# Autodesk Inventor assembly: brace
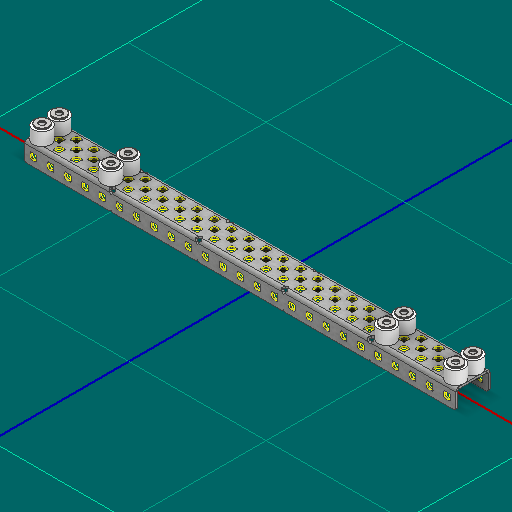
[picture p0: Inventor's stored thumbnail of the model, 512x512]
Saved by Autodesk Inventor 2025 (Build 290162000, 162)
## iProperties
Created: 2024-10-07
Part Number: brace
Document SubType Name: Assembly
Designer: averey
Author: averey
## Documents named in this file (7)
- C:\Users\avere\vex_robotics_high_stakes\hardware\cad\bots\high_stakes_v2\chassis\brace.iam
- C:\Users\avere\vex_robotics_high_stakes\hardware\cad\robpros_cad_lib\Structure\C Channel\Aluminum 1x2x1\Alu C 1x2x1x25.ipt
- C:\Users\avere\vex_robotics_high_stakes\hardware\cad\VEX-CAD-Inventor\Motion\Spacers\Spacer Nylon .500 OD\NSpacer White .500 OD x .375.ipt
- C:\Users\avere\vex_robotics_high_stakes\hardware\cad\VEX-CAD-Inventor\Motion\Spacers\Spacer Nylon .500 OD.ipt
- C:\Users\avere\vex_robotics_high_stakes\hardware\cad\VEX-CAD-Inventor\Motion\Spacers\Washer Steel\SWasher .375 OD x .031250.ipt
- C:\Users\avere\vex_robotics_high_stakes\hardware\cad\VEX-CAD-Inventor\Motion\Spacers\Washer Steel.ipt
- C:\Users\avere\vex_robotics_high_stakes\hardware\cad\VEX-CAD-Inventor\Motion\Spacers\Washer Steel\SWasher .375 OD x .015625.ipt
## Components (25 placed, 4 different names)
1. Alu C 1x2x1x25:1 — Mate:1, Insert:6, Insert:9, Insert:12, Insert:15, Insert:18, Insert:23, Insert:24
2. NSpacer White .500 OD x .375:1 — Insert:6
3. SWasher .375 OD x .031250:1
4. SWasher .375 OD x .015625:2
5. NSpacer White .500 OD x .375:2
6. SWasher .375 OD x .031250:3
7. SWasher .375 OD x .015625:4
8. NSpacer White .500 OD x .375:3 — Insert:9
9. SWasher .375 OD x .031250:5
10. SWasher .375 OD x .015625:6
11. NSpacer White .500 OD x .375:4 — Insert:12
12. SWasher .375 OD x .031250:7
13. SWasher .375 OD x .015625:8
14. NSpacer White .500 OD x .375:5 — Insert:15
15. SWasher .375 OD x .031250:9
16. SWasher .375 OD x .015625:10
17. NSpacer White .500 OD x .375:6 — Insert:18
18. SWasher .375 OD x .031250:11
19. SWasher .375 OD x .015625:12
20. NSpacer White .500 OD x .375:7 — Insert:24
21. SWasher .375 OD x .031250:13
22. SWasher .375 OD x .015625:14
23. NSpacer White .500 OD x .375:8 — Insert:23
24. SWasher .375 OD x .031250:15
25. SWasher .375 OD x .015625:16
## Relationships (25: Insert 24, Mate 1)
- [Insert]: NSpacer White .500 OD x .375:1 ↔ SWasher .375 OD x .031250:1
- [Insert]: SWasher .375 OD x .031250:1 ↔ SWasher .375 OD x .015625:2
- [Insert]: NSpacer White .500 OD x .375:2 ↔ SWasher .375 OD x .031250:3
- [Insert]: SWasher .375 OD x .031250:3 ↔ SWasher .375 OD x .015625:4
- [Insert]: Alu C 1x2x1x25:1 ↔ NSpacer White .500 OD x .375:2
- Mate:1: Alu C 1x2x1x25:1
- Insert:6: Alu C 1x2x1x25:1 ↔ NSpacer White .500 OD x .375:1
- [Insert]: NSpacer White .500 OD x .375:3 ↔ SWasher .375 OD x .031250:5
- [Insert]: SWasher .375 OD x .031250:5 ↔ SWasher .375 OD x .015625:6
- Insert:9: Alu C 1x2x1x25:1 ↔ NSpacer White .500 OD x .375:3
- [Insert]: NSpacer White .500 OD x .375:4 ↔ SWasher .375 OD x .031250:7
- [Insert]: SWasher .375 OD x .031250:7 ↔ SWasher .375 OD x .015625:8
- Insert:12: Alu C 1x2x1x25:1 ↔ NSpacer White .500 OD x .375:4
- [Insert]: NSpacer White .500 OD x .375:5 ↔ SWasher .375 OD x .031250:9
- [Insert]: SWasher .375 OD x .031250:9 ↔ SWasher .375 OD x .015625:10
- Insert:15: Alu C 1x2x1x25:1 ↔ NSpacer White .500 OD x .375:5
- [Insert]: NSpacer White .500 OD x .375:6 ↔ SWasher .375 OD x .031250:11
- [Insert]: SWasher .375 OD x .031250:11 ↔ SWasher .375 OD x .015625:12
- Insert:18: Alu C 1x2x1x25:1 ↔ NSpacer White .500 OD x .375:6
- [Insert]: NSpacer White .500 OD x .375:7 ↔ SWasher .375 OD x .031250:13
- [Insert]: SWasher .375 OD x .031250:13 ↔ SWasher .375 OD x .015625:14
- [Insert]: NSpacer White .500 OD x .375:8 ↔ SWasher .375 OD x .031250:15
- [Insert]: SWasher .375 OD x .031250:15 ↔ SWasher .375 OD x .015625:16
- Insert:23: Alu C 1x2x1x25:1 ↔ NSpacer White .500 OD x .375:8
- Insert:24: Alu C 1x2x1x25:1 ↔ NSpacer White .500 OD x .375:7
## Named parameters: d69_d66 = 0 mm, d70_d67 = 0 mm, d7_d69_d66 = 0 mm, d8_d70_d67 = 0 mm, d10_d69_d66 = 0 mm, d11_d70_d67 = 0 mm, d13_d69_d66 = 0 mm, d14_d70_d67 = 0 mm, d16_d69_d66 = 0 mm, d17_d70_d67 = 0 mm, d19_d69_d66 = 0 mm, d20_d70_d67 = 0 mm, d21_d69_d66 = 0 mm, d22_d70_d67 = 0 mm
